# Autodesk Inventor assembly: DinningTableSquare
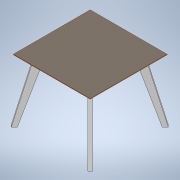
[picture p0: Inventor's stored thumbnail of the model, 180x180]
Saved by Autodesk Inventor 2022 (Build 260153000, 153)
## iProperties
Created: 2022-01-15
Part Number: DinningTableSquare
Document SubType Name: Assembly
Designer: dangl
Author: dangl
## Documents named in this file (4)
- C:\Users\dangl\Documents\WoodWork\BreakfastTable\DinningTableSquare.iam
- C:\Users\dangl\Documents\WoodWork\BreakfastTable\TableTop.ipt
- C:\Users\dangl\Documents\WoodWork\BreakfastTable\Leg.ipt
- C:\Users\dangl\Documents\WoodWork\BreakfastTable\LegConnector_1.ipt
## Components (7 placed, 3 different names)
1. TableTop:1 — Mate:3, Mate:5, Mate:12
2. Leg:1 — Flush:3, Mate:3, Mate:4
3. LegConnector_1:1 — Mate:1, Flush:2, Flush:3, Mate:4, Mate:5, Flush:8, Mate:11
4. Leg:2 — Mate:1, Flush:2, Flush:8
5. Leg:3 — Flush:6
6. LegConnector_1:2 — Flush:6, Flush:7, Mate:9, Mate:12
7. Leg:4 — Flush:7
## Relationships (20: Mate 11, Flush 7, Angle 2)
- Mate:1: LegConnector_1:1 ↔ Leg:2
- Flush:2: LegConnector_1:1 ↔ Leg:2
- Flush:3: Leg:1 ↔ LegConnector_1:1
- Mate:3: TableTop:1 ↔ Leg:1
- Mate:4: Leg:1 ↔ LegConnector_1:1
- Mate:5: TableTop:1 ↔ LegConnector_1:1
- [Mate]: LegConnector_1:2 ↔ Leg:4
- [Flush]: LegConnector_1:2 ↔ Leg:4
- [Flush]: Leg:3 ↔ LegConnector_1:2
- [Mate]: Leg:3 ↔ LegConnector_1:2
- Flush:6: Leg:3 ↔ LegConnector_1:2
- Flush:7: LegConnector_1:2 ↔ Leg:4
- Mate:8
- Angle:1 (45 deg)
- Mate:9: LegConnector_1:2
- Mate:10
- Angle:2 (-45 deg)
- Flush:8: LegConnector_1:1 ↔ Leg:2
- Mate:11: LegConnector_1:1
- Mate:12: TableTop:1 ↔ LegConnector_1:2
## Named parameters: d8_d3 = 0 mm, d9_d4 = 0 mm, d10_d6 = 0 mm, d11_d1 = 0 mm
